# Autodesk Inventor assembly: Assy_upper_plate
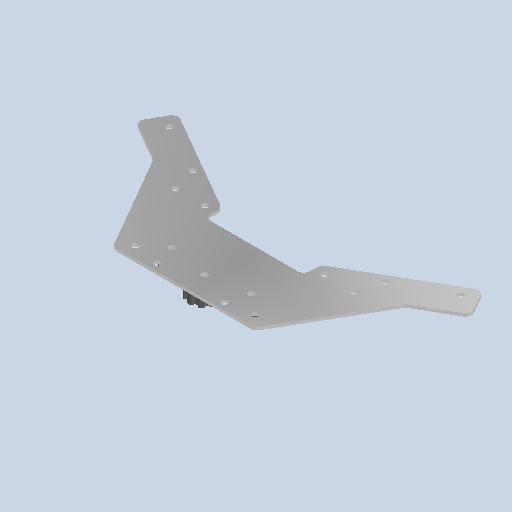
[picture p0: Inventor's stored thumbnail of the model, 512x512]
Saved by Autodesk Inventor 2024.1 (Build 281209000, 209)
## iProperties
Created: 2025-04-23
Part Number: Assy_upper_plate
Document SubType Name: Assembly
Designer: hibik
Author: hibik
## Documents named in this file (5)
- C:\Users\hibik\Documents\Robomech\RESCUE\ORCA\hard\fork\Assy_upper_plate.iam
- C:\Users\hibik\Documents\Robomech\RESCUE\ORCA\hard\fork\upper_plate.ipt
- C:\Users\hibik\Documents\Robomech\RESCUE\ORCA\hard\fork\belt_roller_outside.ipt
- C:\Users\hibik\Documents\Robomech\RESCUE\ORCA\hard\fork\belt_geared_roller.ipt
- C:\Users\hibik\Documents\Robomech\RESCUE\ORCA\hard\std_parts\bearing_3_6_2.5_noscrew.ipt
## Components (10 placed, 4 different names)
1. upper_plate:1 — 挿入:5, 挿入:6, 挿入:9
2. belt_roller_outside:1 — 挿入:1, 挿入:2
3. belt_geared_roller:1 — 挿入:3, 挿入:4
4. bearing_3_6_2.5_noscrew:1 — 挿入:3, 挿入:5
5. bearing_3_6_2.5_noscrew:2 — 挿入:4
6. bearing_3_6_2.5_noscrew:3 — 挿入:1
7. bearing_3_6_2.5_noscrew:4 — 挿入:2, 挿入:6
8. belt_roller_outside:2
9. bearing_3_6_2.5_noscrew:5
10. bearing_3_6_2.5_noscrew:6 — 挿入:9
## Relationships (9: Insert 9)
- 挿入:1 [Insert]: belt_roller_outside:1 ↔ bearing_3_6_2.5_noscrew:3
- 挿入:2 [Insert]: belt_roller_outside:1 ↔ bearing_3_6_2.5_noscrew:4
- 挿入:3 [Insert]: belt_geared_roller:1 ↔ bearing_3_6_2.5_noscrew:1
- 挿入:4 [Insert]: belt_geared_roller:1 ↔ bearing_3_6_2.5_noscrew:2
- 挿入:5 [Insert]: upper_plate:1 ↔ bearing_3_6_2.5_noscrew:1
- 挿入:6 [Insert]: upper_plate:1 ↔ bearing_3_6_2.5_noscrew:4
- [Insert]: belt_roller_outside:2 ↔ bearing_3_6_2.5_noscrew:5
- [Insert]: belt_roller_outside:2 ↔ bearing_3_6_2.5_noscrew:6
- 挿入:9 [Insert]: upper_plate:1 ↔ bearing_3_6_2.5_noscrew:6
## Named parameters: d6_d0 = 0 mm, d7_d1 = 0 mm
